# Autodesk Inventor assembly: 膝_1_1
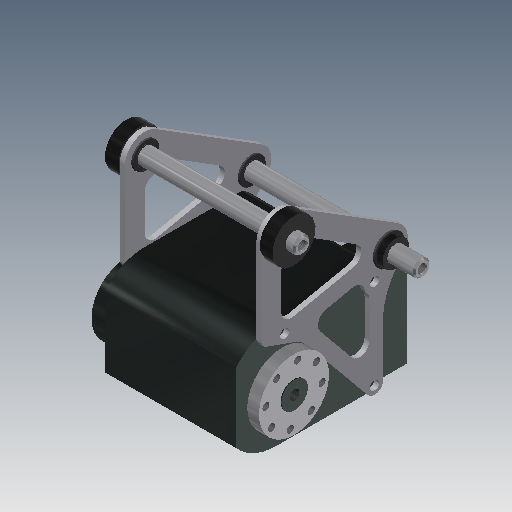
[picture p0: Inventor's stored thumbnail of the model, 512x512]
Saved by Autodesk Inventor 2017.3 (Build 213256000, 256)
## iProperties
Created: 2016-04-27
Part Number: 膝_1_1
Document SubType Name: Assembly
Designer: hiroaki
Mass: 133.749 g
Surface Area: 221.612 cm^2
Volume: 63.598 cm^3
Density: 2.10304 g/cm^3
Author: hiroaki
## Documents named in this file (12)
- C:\Users\haya\Desktop\GankenKun0_5\下半身\膝\膝_1_1_MIR.iam
- C:\Users\haya\Desktop\GankenKun0_5\既製品\B3M11xx.ipt
- C:\Users\haya\Desktop\GankenKun0_5\下半身\膝\膝_メインフレーム_1_1.ipt
- C:\Users\haya\Desktop\GankenKun0_5\下半身\膝\膝_メインフレーム_1_1_MIR.ipt
- C:\Users\haya\Desktop\GankenKun0_5\既製品\free_horn.ipt
- C:\Users\haya\Desktop\GankenKun0_5\下半身\リンク\スペーサ\膝_同軸_スペーサ_1_4.ipt
- C:\Users\haya\Desktop\GankenKun0_5\下半身\リンク\スペーサ\膝_同軸_スペーサ_1_5.ipt
- C:\Users\haya\Desktop\GankenKun0_5\既製品\NSK_RB_MF85ZZ\MF85ZZ.iam
- C:\Users\haya\Desktop\GankenKun0_5\既製品\SETF5-63_5-M3-N3.ipt
- C:\Users\haya\Desktop\GankenKun0_5\既製品\SETF5-55_5-M3-N3.ipt
- C:\Users\haya\Desktop\GankenKun0_5\既製品\LL-5208-10.ipt
- C:\Users\haya\Desktop\GankenKun0_5\既製品\LL-5208-08.ipt
## Components (16 placed, 11 different names)
1. B3M11xx:1 — 挿入:13, 挿入:18, 挿入:19
2. 膝_メインフレーム_1_1:1 — 挿入:19, 挿入:24, フラッシュ:1, 挿入:26
3. 膝_メインフレーム_1_1_MIR:1 — 挿入:18, 挿入:25, 挿入:28
4. free_horn:1 — 挿入:13
5. 膝_同軸_スペーサ_1_4:1 — 挿入:27
6. 膝_同軸_スペーサ_1_5:1 — 挿入:29, メイト:2, フラッシュ:2
7. MF85ZZ:1 [sub-assembly] — 挿入:24, 挿入:30
8. MF85ZZ:2 [sub-assembly] — 挿入:25, メイト:1, 挿入:31
9. SETF5-63_5-M3-N3:1 — メイト:1, フラッシュ:1
10. SETF5-55_5-M3-N3:1 — メイト:2, メイト:3, フラッシュ:2
11. MF85ZZ:3 [sub-assembly] — 挿入:26, 挿入:27, メイト:3
12. MF85ZZ:4 [sub-assembly] — 挿入:28, 挿入:29
13. LL-5208-10:1 — 挿入:31, 挿入:33
14. LL-5208-10:2 — 挿入:30, 挿入:32
15. LL-5208-08:1 — 挿入:32
16. LL-5208-08:2 — 挿入:33
## Relationships (18: Insert 13, Mate 3, Flush 2)
- 挿入:13 [Insert]: B3M11xx:1 ↔ free_horn:1
- 挿入:18 [Insert]: B3M11xx:1 ↔ 膝_メインフレーム_1_1_MIR:1
- 挿入:19 [Insert]: B3M11xx:1 ↔ 膝_メインフレーム_1_1:1
- 挿入:24 [Insert]: 膝_メインフレーム_1_1:1 ↔ MF85ZZ:1
- 挿入:25 [Insert]: 膝_メインフレーム_1_1_MIR:1 ↔ MF85ZZ:2
- メイト:1 [Mate]: MF85ZZ:2 ↔ SETF5-63_5-M3-N3:1
- フラッシュ:1 [Flush] (-10.4 mm): 膝_メインフレーム_1_1:1 ↔ SETF5-63_5-M3-N3:1
- 挿入:26 [Insert]: 膝_メインフレーム_1_1:1 ↔ MF85ZZ:3
- 挿入:27 [Insert]: 膝_同軸_スペーサ_1_4:1 ↔ MF85ZZ:3
- 挿入:28 [Insert]: 膝_メインフレーム_1_1_MIR:1 ↔ MF85ZZ:4
- 挿入:29 [Insert]: 膝_同軸_スペーサ_1_5:1 ↔ MF85ZZ:4
- メイト:2 [Mate]: 膝_同軸_スペーサ_1_5:1 ↔ SETF5-55_5-M3-N3:1
- メイト:3 [Mate]: SETF5-55_5-M3-N3:1 ↔ MF85ZZ:3
- フラッシュ:2 [Flush] (-2.6 mm): 膝_同軸_スペーサ_1_5:1 ↔ SETF5-55_5-M3-N3:1
- 挿入:30 [Insert]: MF85ZZ:1 ↔ LL-5208-10:2
- 挿入:31 [Insert]: MF85ZZ:2 ↔ LL-5208-10:1
- 挿入:32 [Insert]: LL-5208-10:2 ↔ LL-5208-08:1
- 挿入:33 [Insert]: LL-5208-10:1 ↔ LL-5208-08:2
